# Autodesk Inventor assembly: encoder_m
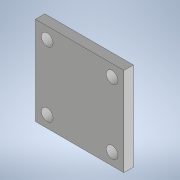
[picture p0: Inventor's stored thumbnail of the model, 180x180]
Saved by Autodesk Inventor 2020 (Build 240168000, 168)
## iProperties
Created: 2019-05-15
Part Number: encoder_m
Document SubType Name: Assembly
Designer: psrob
Author: psrob
## Documents named in this file (3)
- E:\projects-2\project dog gen2\hardware\encoder_m.iam
- E:\projects-2\project dog gen2\hardware\encoder_pcb.ipt
- E:\projects-2\project dog gen2\hardware\as5600.ipt
## Components (2 placed, 2 different names)
1. encoder_pcb:1 — Mate:1, Flush:1, Flush:2
2. as5600:1 — Mate:1, Flush:1, Flush:2
## Relationships (3: Flush 2, Mate 1)
- Mate:1: encoder_pcb:1 ↔ as5600:1
- Flush:1 (5 mm): encoder_pcb:1 ↔ as5600:1
- Flush:2 (4.5 mm): encoder_pcb:1 ↔ as5600:1
